# Autodesk Inventor assembly: gripper manufacturing layout
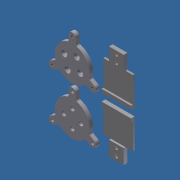
[picture p0: Inventor's stored thumbnail of the model, 180x180]
Saved by Autodesk Inventor 2012 (Build 160160000, 160)
## iProperties
Created: 2012-08-06
Part Number: gripper manufacturing layout
Document SubType Name: Assembly
Designer: Edward
Author: Edward
## Documents named in this file (4)
- C:\Users\Edward\Documents\masters\CAD\Gripper\gripper manufacturing layout.iam
- C:\Users\Edward\Documents\masters\CAD\Gripper\gripper plate.ipt
- C:\Users\Edward\Documents\masters\CAD\Gripper\IRB120 plate.ipt
- C:\Users\Edward\Documents\masters\CAD\Gripper\gripper jaw extension.ipt
## Components (4 placed, 3 different names)
1. gripper plate:1 — Flush:1, Flush:2, Mate:4, Flush:6
2. IRB120 plate:1 — Flush:1, Mate:4, Flush:6
3. gripper jaw extension:1 — Flush:3, Flush:4, Flush:1
4. gripper jaw extension:2 — Flush:2, Flush:3, Flush:4, Flush:1
## Relationships (7: Flush 6, Mate 1)
- Flush:1: gripper plate:1 ↔ IRB120 plate:1
- Flush:2: gripper plate:1 ↔ gripper jaw extension:2
- Flush:3: gripper jaw extension:1 ↔ gripper jaw extension:2
- Flush:4 (-88.9 mm): gripper jaw extension:1 ↔ gripper jaw extension:2
- Flush:1: gripper jaw extension:1 ↔ gripper jaw extension:2
- Mate:4 (82.55 mm): gripper plate:1 ↔ IRB120 plate:1
- Flush:6: gripper plate:1 ↔ IRB120 plate:1
